# Autodesk Inventor assembly: Gas_Burner_Assembly
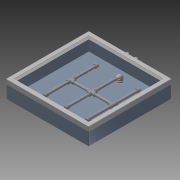
[picture p0: Inventor's stored thumbnail of the model, 180x180]
Saved by Autodesk Inventor 2014 (Build 180170000, 170)
## iProperties
Created: 2016-08-25
Part Number: Gas_Burner_Assembly
Document SubType Name: Assembly
Designer: jmw3
Author: jmw3
## Documents named in this file (10)
- F:\NIST\Project_Files\FFT_Projects\UL_Drawings\Gas_Burner\Inventor_Parts\Gas_Burner_Assembly.iam
- F:\NIST\Project_Files\FFT_Projects\UL_Drawings\Gas_Burner\Inventor_Parts\Propane Burner Base.ipt
- F:\NIST\Project_Files\FFT_Projects\UL_Drawings\Gas_Burner\Inventor_Parts\1in_SS_2in_long_pipe.ipt
- F:\NIST\Project_Files\FFT_Projects\UL_Drawings\Gas_Burner\Inventor_Parts\1 in to .5 in elbow reducer.ipt
- F:\NIST\Project_Files\FFT_Projects\UL_Drawings\Gas_Burner\Inventor_Parts\0.5in_SS_6in_long_pipe.ipt
- F:\NIST\Project_Files\FFT_Projects\UL_Drawings\Gas_Burner\Inventor_Parts\0.5in_SS_Cross.ipt
- F:\NIST\Project_Files\FFT_Projects\UL_Drawings\Gas_Burner\Inventor_Parts\0.5in_SS_8in_long_pipe.ipt
- F:\NIST\Project_Files\FFT_Projects\UL_Drawings\Gas_Burner\Inventor_Parts\0.5in_SS_Tee.ipt
- F:\NIST\Project_Files\FFT_Projects\UL_Drawings\Gas_Burner\Inventor_Parts\0.5in_pipe_cap.ipt
- F:\NIST\Project_Files\FFT_Projects\UL_Drawings\Gas_Burner\Inventor_Parts\Propane Burner Lid.ipt
## Components (20 placed, 9 different names)
1. Propane Burner Base:1 — Mate:1, Mate:2, Mate:3, Mate:5, Mate:6, Mate:44, Mate:45, Mate:46
2. 1in_SS_2in_long_pipe:1 — Mate:1, Mate:2, Mate:3, Mate:4
3. 1 in to .5 in elbow reducer:1 — Mate:4, Mate:5, Mate:6, Mate:7, Mate:8, Mate:11, Mate:12
4. 0.5in_SS_8in_long_pipe:1 — Mate:7, Mate:8, Mate:9, Mate:10, Mate:12
5. 0.5in_SS_Cross:1 — Mate:9, Mate:10, Mate:11, Mate:13, Mate:14, Mate:15, Mate:16, Mate:17, Flush:1, Mate:26, Mate:32
6. 0.5in_SS_6in_long_pipe:1 — Mate:16, Mate:17, Flush:1, Mate:19, Mate:20
7. 0.5in_SS_6in_long_pipe:2 — Mate:13, Mate:14, Mate:15, Mate:18, Mate:21, Mate:22, Mate:23
8. 0.5in_SS_Tee:1 — Mate:21, Mate:22, Mate:23, Mate:24, Mate:25, Mate:31, Mate:33
9. 0.5in_SS_Tee:2 — Mate:18, Mate:19, Mate:20, Mate:27, Mate:28, Mate:29, Mate:30
10. 0.5in_SS_8in_long_pipe:2 — Mate:24, Mate:33, Mate:34, Mate:41
11. 0.5in_SS_8in_long_pipe:3 — Mate:25, Mate:31, Mate:37, Mate:40
12. 0.5in_SS_8in_long_pipe:4 — Mate:26, Mate:32, Mate:35, Mate:42
13. 0.5in_SS_8in_long_pipe:5 — Mate:27, Mate:29, Mate:36, Mate:43
14. 0.5in_SS_8in_long_pipe:6 — Mate:28, Mate:30, Mate:38, Mate:39
15. 0.5in_pipe_cap:1 — Mate:34, Mate:41
16. 0.5in_pipe_cap:2 — Mate:35, Mate:42
17. 0.5in_pipe_cap:3 — Mate:36, Mate:43
18. 0.5in_pipe_cap:4 — Mate:37, Mate:40
19. 0.5in_pipe_cap:5 — Mate:38, Mate:39
20. Propane Burner Lid:1 — Mate:44, Mate:45, Mate:46
## Relationships (47: Mate 46, Flush 1)
- Mate:1: Propane Burner Base:1 ↔ 1in_SS_2in_long_pipe:1
- Mate:2: Propane Burner Base:1 ↔ 1in_SS_2in_long_pipe:1
- Mate:3 (-25.4 mm): Propane Burner Base:1 ↔ 1in_SS_2in_long_pipe:1
- Mate:4: 1in_SS_2in_long_pipe:1 ↔ 1 in to .5 in elbow reducer:1
- Mate:5: Propane Burner Base:1 ↔ 1 in to .5 in elbow reducer:1
- Mate:6: Propane Burner Base:1 ↔ 1 in to .5 in elbow reducer:1
- Mate:7: 1 in to .5 in elbow reducer:1 ↔ 0.5in_SS_8in_long_pipe:1
- Mate:8: 1 in to .5 in elbow reducer:1 ↔ 0.5in_SS_8in_long_pipe:1
- Mate:9: 0.5in_SS_8in_long_pipe:1 ↔ 0.5in_SS_Cross:1
- Mate:10: 0.5in_SS_8in_long_pipe:1 ↔ 0.5in_SS_Cross:1
- Mate:11: 1 in to .5 in elbow reducer:1 ↔ 0.5in_SS_Cross:1
- Mate:12: 1 in to .5 in elbow reducer:1 ↔ 0.5in_SS_8in_long_pipe:1
- Mate:13: 0.5in_SS_Cross:1 ↔ 0.5in_SS_6in_long_pipe:2
- Mate:14: 0.5in_SS_Cross:1 ↔ 0.5in_SS_6in_long_pipe:2
- Mate:15: 0.5in_SS_Cross:1 ↔ 0.5in_SS_6in_long_pipe:2
- Mate:16: 0.5in_SS_Cross:1 ↔ 0.5in_SS_6in_long_pipe:1
- Mate:17: 0.5in_SS_Cross:1 ↔ 0.5in_SS_6in_long_pipe:1
- Flush:1: 0.5in_SS_Cross:1 ↔ 0.5in_SS_6in_long_pipe:1
- Mate:18: 0.5in_SS_6in_long_pipe:2 ↔ 0.5in_SS_Tee:2
- Mate:19: 0.5in_SS_6in_long_pipe:1 ↔ 0.5in_SS_Tee:2
- Mate:20: 0.5in_SS_6in_long_pipe:1 ↔ 0.5in_SS_Tee:2
- Mate:21: 0.5in_SS_6in_long_pipe:2 ↔ 0.5in_SS_Tee:1
- Mate:22: 0.5in_SS_6in_long_pipe:2 ↔ 0.5in_SS_Tee:1
- Mate:23: 0.5in_SS_6in_long_pipe:2 ↔ 0.5in_SS_Tee:1
- Mate:24: 0.5in_SS_Tee:1 ↔ 0.5in_SS_8in_long_pipe:2
- Mate:25: 0.5in_SS_Tee:1 ↔ 0.5in_SS_8in_long_pipe:3
- Mate:26: 0.5in_SS_Cross:1 ↔ 0.5in_SS_8in_long_pipe:4
- Mate:27: 0.5in_SS_Tee:2 ↔ 0.5in_SS_8in_long_pipe:5
- Mate:28: 0.5in_SS_Tee:2 ↔ 0.5in_SS_8in_long_pipe:6
- Mate:29: 0.5in_SS_Tee:2 ↔ 0.5in_SS_8in_long_pipe:5
- Mate:30: 0.5in_SS_Tee:2 ↔ 0.5in_SS_8in_long_pipe:6
- Mate:31: 0.5in_SS_Tee:1 ↔ 0.5in_SS_8in_long_pipe:3
- Mate:32: 0.5in_SS_Cross:1 ↔ 0.5in_SS_8in_long_pipe:4
- Mate:33: 0.5in_SS_Tee:1 ↔ 0.5in_SS_8in_long_pipe:2
- Mate:34: 0.5in_SS_8in_long_pipe:2 ↔ 0.5in_pipe_cap:1
- Mate:35: 0.5in_SS_8in_long_pipe:4 ↔ 0.5in_pipe_cap:2
- Mate:36: 0.5in_SS_8in_long_pipe:5 ↔ 0.5in_pipe_cap:3
- Mate:37: 0.5in_SS_8in_long_pipe:3 ↔ 0.5in_pipe_cap:4
- Mate:38: 0.5in_SS_8in_long_pipe:6 ↔ 0.5in_pipe_cap:5
- Mate:39: 0.5in_SS_8in_long_pipe:6 ↔ 0.5in_pipe_cap:5
- Mate:40: 0.5in_SS_8in_long_pipe:3 ↔ 0.5in_pipe_cap:4
- Mate:41: 0.5in_SS_8in_long_pipe:2 ↔ 0.5in_pipe_cap:1
- Mate:42: 0.5in_SS_8in_long_pipe:4 ↔ 0.5in_pipe_cap:2
- Mate:43: 0.5in_SS_8in_long_pipe:5 ↔ 0.5in_pipe_cap:3
- Mate:44: Propane Burner Base:1 ↔ Propane Burner Lid:1
- Mate:45: Propane Burner Base:1 ↔ Propane Burner Lid:1
- Mate:46: Propane Burner Base:1 ↔ Propane Burner Lid:1
